# Autodesk Inventor assembly: CycloidalJoint1
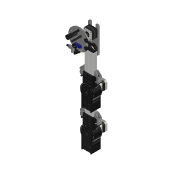
[picture p0: Inventor's stored thumbnail of the model, 180x180]
Saved by Autodesk Inventor 2020.3 (Build 243373000, 373)
## iProperties
Created: 2021-08-10
Part Number: CycloidalJoint1
Document SubType Name: Assembly
Designer: justi
Mass: 1624.46 g
Surface Area: 3704.2 cm^2
Volume: 788.977 cm^3
Density: 2.05895 g/cm^3
Author: justi
## Documents named in this file (26)
- F:\UQ Engineering\2021 ~ 5th Year\Semester 2\METR4911-THESIS\FarmBot CAD\FarmBotV1\CycloidalJoint1.iam
- F:\UQ Engineering\2021 ~ 5th Year\Semester 2\METR4911-THESIS\FarmBot CAD\FarmBotV1\CycloidalJoint\simple_cyc_nema17\stepper_top_new.ipt
- F:\UQ Engineering\2021 ~ 5th Year\Semester 2\METR4911-THESIS\FarmBot CAD\FarmBotV1\LinearRail\20x40x40mm.ipt
- F:\UQ Engineering\2021 ~ 5th Year\Semester 2\METR4911-THESIS\FarmBot CAD\FarmBotV1\CycloidalJoint\simple_cyc_nema17\Motor_paso.ipt
- F:\UQ Engineering\2021 ~ 5th Year\Semester 2\METR4911-THESIS\FarmBot CAD\FarmBotV1\CycloidalJoint\Cycloid CAD\65x50x7 bearing.ipt
- F:\UQ Engineering\2021 ~ 5th Year\Semester 2\METR4911-THESIS\FarmBot CAD\FarmBotV1\CycloidalJoint\old-new-cycloidal\3mm_pin.ipt
- F:\UQ Engineering\2021 ~ 5th Year\Semester 2\METR4911-THESIS\FarmBot CAD\FarmBotV1\CycloidalJoint\simple_cyc_nema17\ecc_shaft.ipt
- F:\UQ Engineering\2021 ~ 5th Year\Semester 2\METR4911-THESIS\FarmBot CAD\FarmBotV1\CycloidalJoint\Cycloid CAD\18x12x4 bearing.ipt
- F:\UQ Engineering\2021 ~ 5th Year\Semester 2\METR4911-THESIS\FarmBot CAD\FarmBotV1\CycloidalJoint\bldc_capstan\27x20x4 bearing.ipt
- F:\UQ Engineering\2021 ~ 5th Year\Semester 2\METR4911-THESIS\FarmBot CAD\FarmBotV1\CycloidalJoint\simple_cyc_nema17\bottom_clip.ipt
- F:\UQ Engineering\2021 ~ 5th Year\Semester 2\METR4911-THESIS\FarmBot CAD\FarmBotV1\CycloidalJoint\simple_cyc_nema17\top_clip.ipt
- F:\UQ Engineering\2021 ~ 5th Year\Semester 2\METR4911-THESIS\FarmBot CAD\FarmBotV1\CycloidalJoint\Cycloid CAD\15x10x4 bearing.ipt
- F:\UQ Engineering\2021 ~ 5th Year\Semester 2\METR4911-THESIS\FarmBot CAD\FarmBotV1\CycloidalJoint\simple_cyc_nema17\Main_equation_step_simple_upper.ipt
- F:\UQ Engineering\2021 ~ 5th Year\Semester 2\METR4911-THESIS\FarmBot CAD\FarmBotV1\CycloidalJoint\simple_cyc_nema17\Main_equation_step_simple.ipt
- F:\UQ Engineering\2021 ~ 5th Year\Semester 2\METR4911-THESIS\FarmBot CAD\FarmBotV1\CycloidalJoint\simple_cyc_nema17\stepper_bottom_new.ipt
- F:\UQ Engineering\2021 ~ 5th Year\Semester 2\METR4911-THESIS\FarmBot CAD\FarmBotV1\CycloidalJoint\simple_cyc_nema17\output_new.ipt
- F:\UQ Engineering\2021 ~ 5th Year\Semester 2\METR4911-THESIS\FarmBot CAD\FarmBotV1\LinearRail\20x40_Link1.ipt
- F:\UQ Engineering\2021 ~ 5th Year\Semester 2\METR4911-THESIS\FarmBot CAD\FarmBotV1\LinearRail\20x40_Link3.ipt
- F:\UQ Engineering\2021 ~ 5th Year\Semester 2\METR4911-THESIS\FarmBot CAD\FarmBotV1\New_End_Effector_Assembly.iam
- F:\UQ Engineering\2021 ~ 5th Year\Semester 2\METR4911-THESIS\FarmBot CAD\FarmBotV1\CYC_limitswitch assembly.iam
- F:\UQ Engineering\2021 ~ 5th Year\Semester 2\METR4911-THESIS\FarmBot CAD\FarmBotV1\CycloidalJoint1\AIP\FEA\drtrevt6o.fins
- F:\UQ Engineering\2021 ~ 5th Year\Semester 2\METR4911-THESIS\FarmBot CAD\FarmBotV1\CycloidalJoint1\AIP\FEA\drtrevt6o.fsat
- F:\UQ Engineering\2021 ~ 5th Year\Semester 2\METR4911-THESIS\FarmBot CAD\FarmBotV1\CycloidalJoint1\AIP\FEA\drtrevt6o.ftes
- F:\UQ Engineering\2021 ~ 5th Year\Semester 2\METR4911-THESIS\FarmBot CAD\FarmBotV1\CycloidalJoint1\AIP\FEA\drtrevt6o.fwiz
- F:\UQ Engineering\2021 ~ 5th Year\Semester 2\METR4911-THESIS\FarmBot CAD\FarmBotV1\CycloidalJoint1\AIP\FEA\drtrevu0w.fmsh
- F:\UQ Engineering\2021 ~ 5th Year\Semester 2\METR4911-THESIS\FarmBot CAD\FarmBotV1\CycloidalJoint1\AIP\FEA\drtrevu0x.fres
## Components (55 placed, 19 different names)
1. stepper_top_new:1 — Mate:6, Mate:7, Mate:8, Mate:9, Mate:10, Mate:11, Mate:12, Mate:13, Flush:1, Mate:14, Mate:15, Mate:17, Mate:18, Mate:19, Mate:20, Mate:21, Mate:22, Mate:23, Mate:54
2. 20x40x40mm:1 — Mate:6, Mate:7, Mate:8
3. Motor_paso:1 — Mate:9, Mate:10, Mate:11, Mate:12, Mate:24, Mate:25
4. 65x50x7 bearing:1 — Mate:13, Flush:1, Mate:50, Mate:55, Flush:9
5. 3mm_pin:1 — Mate:14, Mate:15, Flush:2, Flush:3, Flush:4, Flush:5, Flush:6, Flush:7
6. 18x12x4 bearing:1 — Mate:35, Mate:36
7. 18x12x4 bearing:2 — Mate:33, Mate:34, Mate:36, Mate:48
8. 27x20x4 bearing:1 — Mate:28, Mate:29
9. 27x20x4 bearing:2 — Mate:26, Mate:27, Mate:29, Mate:47, Flush:8
10. bottom_clip:1 — Mate:30, Mate:31, Mate:32, Mate:49
11. top_clip:1 — Mate:41, Mate:44, Mate:45
12. 15x10x4 bearing:1 — Mate:42, Mate:43, Mate:52
13. 3mm_pin:3 — Mate:17, Flush:2
14. 3mm_pin:4 — Mate:18, Flush:3
15. 3mm_pin:5 — Mate:19, Flush:4
16. 3mm_pin:6 — Mate:22, Flush:6
17. 3mm_pin:9 — Mate:23, Flush:5, Mate:46
18. 3mm_pin:10 — Mate:21, Mate:46
19. 3mm_pin:11 — Mate:20, Flush:7
20. ecc_shaft:1 — Mate:24, Mate:25, Mate:26, Mate:27, Mate:28, Mate:30, Mate:31, Mate:32, Mate:33, Mate:34, Mate:35, Mate:41, Mate:42, Mate:43, Mate:44, Mate:45
21. Main_equation_step_simple_upper:1 — Mate:48, Mate:49, Mate:51
22. Main_equation_step_simple:1 — Mate:47, Flush:8
23. 65x50x7 bearing:2 — Mate:50, Mate:51, Mate:53
24. stepper_bottom_new:1 — Mate:52, Mate:53, Mate:54
25. output_new:1 — Mate:55, Flush:9, Mate:57, Mate:58, Mate:59, Mate:117, Mate:120
26. 20x40_Link1:1 — Mate:57, Mate:58, Mate:59, Mate:106, Mate:107, Mate:108, Mate:115, Mate:116, Mate:119, Flush:19
27. stepper_top_new:2 — Mate:106, Mate:107
28. Motor_paso:2
29. 65x50x7 bearing:3
30. 3mm_pin:12
31. 18x12x4 bearing:3
32. 18x12x4 bearing:4
33. 27x20x4 bearing:3
34. 27x20x4 bearing:4
35. bottom_clip:2
36. top_clip:2
37. 15x10x4 bearing:2
38. 3mm_pin:14
39. 3mm_pin:15
40. 3mm_pin:16
41. 3mm_pin:17
42. 3mm_pin:18
43. 3mm_pin:19
44. ecc_shaft:2
45. Main_equation_step_simple_upper:2
46. Main_equation_step_simple:2
47. 65x50x7 bearing:4
48. stepper_bottom_new:2 — Mate:108
49. output_new:2 — Mate:109, Mate:110, Mate:111, Mate:114, Mate:121, Mate:124
50. 20x40_Link3:1 — Mate:109, Mate:110, Mate:111, Mate:112, Mate:113, Mate:122, Mate:123, Mate:125, Flush:20
51. New_End_Effector_Assembly:1 [sub-assembly] — Mate:112, Mate:113, Mate:114
52. CYC_limitswitch assembly:1 [sub-assembly] — Mate:119, Mate:120, Flush:19
53. CYC_limitswitch assembly:2 [sub-assembly] — Mate:115, Mate:116, Mate:117
54. CYC_limitswitch assembly:3 [sub-assembly] — Mate:121, Mate:122, Mate:123
55. CYC_limitswitch assembly:4 [sub-assembly] — Mate:124, Mate:125, Flush:20
## Relationships (127: Mate 108, Flush 19)
- Mate:6: stepper_top_new:1 ↔ 20x40x40mm:1
- Mate:7: stepper_top_new:1 ↔ 20x40x40mm:1
- Mate:8: stepper_top_new:1 ↔ 20x40x40mm:1
- Mate:9: stepper_top_new:1 ↔ Motor_paso:1
- Mate:10: stepper_top_new:1 ↔ Motor_paso:1
- Mate:11: stepper_top_new:1 ↔ Motor_paso:1
- Mate:12: stepper_top_new:1 ↔ Motor_paso:1
- Mate:13: stepper_top_new:1 ↔ 65x50x7 bearing:1
- Flush:1: stepper_top_new:1 ↔ 65x50x7 bearing:1
- Mate:14: stepper_top_new:1 ↔ 3mm_pin:1
- Mate:15: stepper_top_new:1 ↔ 3mm_pin:1
- Mate:17: stepper_top_new:1 ↔ 3mm_pin:3
- Mate:18: stepper_top_new:1 ↔ 3mm_pin:4
- Mate:19: stepper_top_new:1 ↔ 3mm_pin:5
- Mate:20: stepper_top_new:1 ↔ 3mm_pin:11
- Mate:21: stepper_top_new:1 ↔ 3mm_pin:10
- Mate:22: stepper_top_new:1 ↔ 3mm_pin:6
- Mate:23: stepper_top_new:1 ↔ 3mm_pin:9
- Flush:2: 3mm_pin:1 ↔ 3mm_pin:3
- Flush:3: 3mm_pin:1 ↔ 3mm_pin:4
- Flush:4: 3mm_pin:1 ↔ 3mm_pin:5
- Flush:5: 3mm_pin:1 ↔ 3mm_pin:9
- Flush:6: 3mm_pin:1 ↔ 3mm_pin:6
- Flush:7: 3mm_pin:1 ↔ 3mm_pin:11
- Mate:24: Motor_paso:1 ↔ ecc_shaft:1
- Mate:25 (1 mm): Motor_paso:1 ↔ ecc_shaft:1
- Mate:26: 27x20x4 bearing:2 ↔ ecc_shaft:1
- Mate:27: 27x20x4 bearing:2 ↔ ecc_shaft:1
- Mate:28: 27x20x4 bearing:1 ↔ ecc_shaft:1
- Mate:29 (1 mm): 27x20x4 bearing:1 ↔ 27x20x4 bearing:2
- Mate:30: bottom_clip:1 ↔ ecc_shaft:1
- Mate:31: bottom_clip:1 ↔ ecc_shaft:1
- Mate:32: bottom_clip:1 ↔ ecc_shaft:1
- Mate:33: 18x12x4 bearing:2 ↔ ecc_shaft:1
- Mate:34: 18x12x4 bearing:2 ↔ ecc_shaft:1
- Mate:35: 18x12x4 bearing:1 ↔ ecc_shaft:1
- Mate:36 (1 mm): 18x12x4 bearing:1 ↔ 18x12x4 bearing:2
- Mate:41: top_clip:1 ↔ ecc_shaft:1
- Mate:42: 15x10x4 bearing:1 ↔ ecc_shaft:1
- Mate:43: 15x10x4 bearing:1 ↔ ecc_shaft:1
- Mate:44: top_clip:1 ↔ ecc_shaft:1
- Mate:45: top_clip:1 ↔ ecc_shaft:1
- Mate:46: 3mm_pin:9 ↔ 3mm_pin:10
- Mate:47: 27x20x4 bearing:2 ↔ Main_equation_step_simple:1
- Flush:8: 27x20x4 bearing:2 ↔ Main_equation_step_simple:1
- Mate:48: 18x12x4 bearing:2 ↔ Main_equation_step_simple_upper:1
- Mate:49: bottom_clip:1 ↔ Main_equation_step_simple_upper:1
- Mate:50: 65x50x7 bearing:1 ↔ 65x50x7 bearing:2
- Mate:51: Main_equation_step_simple_upper:1 ↔ 65x50x7 bearing:2
- Mate:52: 15x10x4 bearing:1 ↔ stepper_bottom_new:1
- Mate:53: 65x50x7 bearing:2 ↔ stepper_bottom_new:1
- Mate:54: stepper_top_new:1 ↔ stepper_bottom_new:1
- Mate:55: 65x50x7 bearing:1 ↔ output_new:1
- Flush:9: 65x50x7 bearing:1 ↔ output_new:1
- Mate:57: output_new:1 ↔ 20x40_Link1:1
- Mate:58: output_new:1 ↔ 20x40_Link1:1
- Mate:59: output_new:1 ↔ 20x40_Link1:1
- [Mate]: stepper_top_new:2 ↔ Motor_paso:2
- [Mate]: stepper_top_new:2 ↔ Motor_paso:2
- [Mate]: stepper_top_new:2 ↔ Motor_paso:2
- [Mate]: stepper_top_new:2 ↔ Motor_paso:2
- [Mate]: stepper_top_new:2 ↔ 65x50x7 bearing:3
- [Flush]: stepper_top_new:2 ↔ 65x50x7 bearing:3
- [Mate]: stepper_top_new:2 ↔ 3mm_pin:12
- [Mate]: stepper_top_new:2 ↔ 3mm_pin:12
- [Mate]: stepper_top_new:2 ↔ 3mm_pin:14
- [Mate]: stepper_top_new:2 ↔ 3mm_pin:15
- [Mate]: stepper_top_new:2 ↔ 3mm_pin:19
- [Mate]: stepper_top_new:2 ↔ 3mm_pin:18
- [Mate]: stepper_top_new:2 ↔ 3mm_pin:16
- [Mate]: stepper_top_new:2 ↔ 3mm_pin:17
- [Flush]: 3mm_pin:12 ↔ 3mm_pin:14
- [Flush]: 3mm_pin:12 ↔ 3mm_pin:15
- [Flush]: 3mm_pin:12 ↔ 3mm_pin:17
- [Flush]: 3mm_pin:12 ↔ 3mm_pin:16
- [Flush]: 3mm_pin:12 ↔ 3mm_pin:19
- [Mate]: Motor_paso:2 ↔ ecc_shaft:2
- [Mate] (1 mm): Motor_paso:2 ↔ ecc_shaft:2
- [Mate]: 27x20x4 bearing:4 ↔ ecc_shaft:2
- [Mate]: 27x20x4 bearing:4 ↔ ecc_shaft:2
- [Mate]: 27x20x4 bearing:3 ↔ ecc_shaft:2
- [Mate] (1 mm): 27x20x4 bearing:3 ↔ 27x20x4 bearing:4
- [Mate]: bottom_clip:2 ↔ ecc_shaft:2
- [Mate]: bottom_clip:2 ↔ ecc_shaft:2
- [Mate]: bottom_clip:2 ↔ ecc_shaft:2
- [Mate]: 18x12x4 bearing:4 ↔ ecc_shaft:2
- [Mate]: 18x12x4 bearing:4 ↔ ecc_shaft:2
- [Mate]: 18x12x4 bearing:3 ↔ ecc_shaft:2
- [Mate] (1 mm): 18x12x4 bearing:3 ↔ 18x12x4 bearing:4
- [Mate]: top_clip:2 ↔ ecc_shaft:2
- [Mate]: 15x10x4 bearing:2 ↔ ecc_shaft:2
- [Mate]: 15x10x4 bearing:2 ↔ ecc_shaft:2
- [Mate]: top_clip:2 ↔ ecc_shaft:2
- [Mate]: top_clip:2 ↔ ecc_shaft:2
- [Mate]: 3mm_pin:17 ↔ 3mm_pin:18
- [Mate]: 27x20x4 bearing:4 ↔ Main_equation_step_simple:2
- [Flush]: 27x20x4 bearing:4 ↔ Main_equation_step_simple:2
- [Mate]: 18x12x4 bearing:4 ↔ Main_equation_step_simple_upper:2
- [Mate]: bottom_clip:2 ↔ Main_equation_step_simple_upper:2
- [Mate]: 65x50x7 bearing:3 ↔ 65x50x7 bearing:4
- [Mate]: Main_equation_step_simple_upper:2 ↔ 65x50x7 bearing:4
- [Mate]: 15x10x4 bearing:2 ↔ stepper_bottom_new:2
- [Mate]: 65x50x7 bearing:4 ↔ stepper_bottom_new:2
- [Mate]: stepper_top_new:2 ↔ stepper_bottom_new:2
- [Mate]: 65x50x7 bearing:3 ↔ output_new:2
- [Flush]: 65x50x7 bearing:3 ↔ output_new:2
- Mate:106: 20x40_Link1:1 ↔ stepper_top_new:2
- Mate:107: 20x40_Link1:1 ↔ stepper_top_new:2
- Mate:108: 20x40_Link1:1 ↔ stepper_bottom_new:2
- Mate:109: output_new:2 ↔ 20x40_Link3:1
- Mate:110: output_new:2 ↔ 20x40_Link3:1
- Mate:111: output_new:2 ↔ 20x40_Link3:1
- Mate:112: 20x40_Link3:1 ↔ New_End_Effector_Assembly:1
- Mate:113: 20x40_Link3:1 ↔ New_End_Effector_Assembly:1
- Mate:114 (75 mm): output_new:2 ↔ New_End_Effector_Assembly:1
- Mate:115 (5 mm): 20x40_Link1:1 ↔ CYC_limitswitch assembly:2
- Mate:116: 20x40_Link1:1 ↔ CYC_limitswitch assembly:2
- Mate:117: output_new:1 ↔ CYC_limitswitch assembly:2
- Mate:119 (5 mm): 20x40_Link1:1 ↔ CYC_limitswitch assembly:1
- Mate:120: output_new:1 ↔ CYC_limitswitch assembly:1
- Flush:19: 20x40_Link1:1 ↔ CYC_limitswitch assembly:1
- Mate:121: output_new:2 ↔ CYC_limitswitch assembly:3
- Mate:122: 20x40_Link3:1 ↔ CYC_limitswitch assembly:3
- Mate:123 (5 mm): 20x40_Link3:1 ↔ CYC_limitswitch assembly:3
- Mate:124: output_new:2 ↔ CYC_limitswitch assembly:4
- Mate:125 (5 mm): 20x40_Link3:1 ↔ CYC_limitswitch assembly:4
- Flush:20: 20x40_Link3:1 ↔ CYC_limitswitch assembly:4
## Named parameters: d98_d17 = 0 mm, d99_d18 = 0 mm, d100_d19 = 0 mm, d101_d20 = 0 mm, d102_d21 = 0 mm, d103_d23 = 0 mm, d104_d24 = 0 mm, d105_d25 = 0 mm, d107_d84 = 0 mm, d108_d85 = 0 mm, d109_d86 = 0 mm, d110_d87 = 0 mm, d111_d88 = 0 mm, d112_d89 = 0 mm, d113_d90 = 0 mm, d114_d91 = 0 mm, d116_d48 = 0 mm, d117_d49 = 0 mm, d118_d50 = 1 mm, d119_d51 = 0 mm, d120_d52 = 0 mm, d121_d53 = 0 mm, d122_d54 = 1 mm, d123_d55 = 0 mm, d124_d56 = 0 mm, d125_d57 = 0 mm, d126_d58 = 0 mm, d127_d59 = 0 mm, d129_d37 = 0 mm, d130_d38 = 0 mm, d131_d39 = 0 mm, d132_d40 = 0 mm, d133_d41 = 0 mm, d134_d42 = 0 mm, d136_d44 = 0 mm, d137_d45 = 0 mm, d138_d46 = 0 mm, d139_d47 = 0 mm, d140_d60 = 0 mm, d141_d61 = 1 mm, d142_d74 = 0 mm, d143_d75 = 0 mm, d144_d76 = 0 mm, d145_d77 = 0 mm, d146_d78 = 0 mm, d147_d79 = 0 mm, d148_d80 = 0 mm, d149_d81 = 0 mm, d150_d82 = 0 mm, sa_0 = 19600, sa_1 = 981
note: some values were not read from the file. Shown as the stored number, unit unknown: "sa_0", "sa_1".
